# Autodesk Inventor assembly: Lenstube
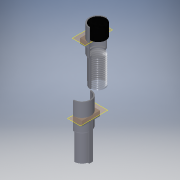
[picture p0: Inventor's stored thumbnail of the model, 180x180]
Saved by Autodesk Inventor 2016 (Build 200138000, 138)
## iProperties
Created: 2016-09-10
Part Number: Lenstube
Material: Generisch
Document SubType Name: Assembly
Designer: Bene
Mass: 21.2233 g
Surface Area: 178.623 cm^2
Volume: 21.2233 cm^3
Density: 1 g/cm^3
Author: Bene
## Documents named in this file (5)
- C:\Users\Bene\Dropbox\Dokumente\OpticalDesign\Beamerscope\Inventor\Beamerscope_r2\Lenstube.iam
- C:\Users\Bene\Dropbox\Dokumente\OpticalDesign\Beamerscope\Inventor\Beamerscope_r2\00_CollectorLens-30mm.ipt
- C:\Users\Bene\Dropbox\Dokumente\OpticalDesign\Beamerscope\Inventor\Beamerscope_r2\01_CondensorLens-16mm.ipt
- C:\Users\Bene\Dropbox\Dokumente\OpticalDesign\Beamerscope\Inventor\Beamerscope_r2\02_Lenstube.ipt
- C:\Users\Bene\Dropbox\Dokumente\OpticalDesign\Beamerscope\Inventor\Beamerscope_r2\02_Lenstube_upper.ipt
## Components (4 placed, 4 different names)
1. 00_CollectorLens-30mm:1
2. 01_CondensorLens-16mm:1
3. 02_Lenstube:1 — Fluchtend:1
4. 02_Lenstube_upper:1 — Fluchtend:1
## Relationships (1: Flush 1)
- Fluchtend:1 [Flush]: 02_Lenstube:1 ↔ 02_Lenstube_upper:1
